# Autodesk Inventor assembly: Shoulder_assembly
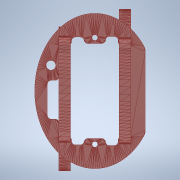
[picture p0: Inventor's stored thumbnail of the model, 180x180]
Saved by Autodesk Inventor 2022 (Build 260153000, 153)
## iProperties
Created: 2023-02-15
Part Number: Shoulder_assembly
Document SubType Name: Assembly
Designer: scott
Author: scott
## Documents named in this file (3)
- C:\Users\scott\OneDrive\Documents\Cat project\Git_repository\Flinders_OpenCat\CAD components\Shoulder_assembly.iam
- C:\Users\scott\OneDrive\Documents\Cat project\Git_repository\Flinders_OpenCat\CAD components\NybbleDIY\Imported Components\Chest_Hips\Chest_Hips.ipt
- C:\Users\scott\OneDrive\Documents\Cat project\Git_repository\Flinders_OpenCat\CAD components\NybbleDIY\Imported Components\Shoulder\Shoulder.ipt
## Components (4 placed, 2 different names)
1. Chest_Hips:1 — Mate:1, Mate:2, Mate:3, Mate:4, Mate:5, Mate:6, Mate:7
2. Chest_Hips:2 — Mate:8, Mate:9, Mate:10
3. Shoulder:1 — Mate:1, Mate:3, Mate:4, Mate:8, Mate:9, Mate:10
4. Shoulder:2 — Mate:2, Mate:5, Mate:6, Mate:7
## Relationships (10: Mate 10)
- Mate:1: Chest_Hips:1 ↔ Shoulder:1
- Mate:2: Chest_Hips:1 ↔ Shoulder:2
- Mate:3: Chest_Hips:1 ↔ Shoulder:1
- Mate:4: Chest_Hips:1 ↔ Shoulder:1
- Mate:5: Chest_Hips:1 ↔ Shoulder:2
- Mate:6: Chest_Hips:1 ↔ Shoulder:2
- Mate:7: Chest_Hips:1 ↔ Shoulder:2
- Mate:8: Chest_Hips:2 ↔ Shoulder:1
- Mate:9: Chest_Hips:2 ↔ Shoulder:1
- Mate:10: Chest_Hips:2 ↔ Shoulder:1
